# Autodesk Inventor assembly: Swingarm
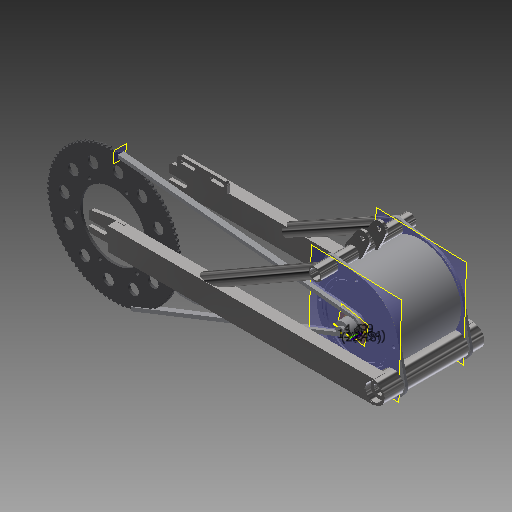
[picture p0: Inventor's stored thumbnail of the model, 512x512]
Saved by Autodesk Inventor 2019.3 (Build 233278000, 278)
## iProperties
Created: 2018-12-13
Part Number: Swingarm
Document SubType Name: Assembly
Designer: eroldan
Author: eroldan
## Documents named in this file (6)
- C:\Users\eroldan\Desktop\3dprojects\OpenEmoto\Swingarm3\Swingarm3.iam
- C:\Users\eroldan\Desktop\3dprojects\OpenEmoto\OtherParts\Denzel4500Motor.iam
- C:\Users\eroldan\Desktop\3dprojects\OpenEmoto\Swingarm3\Swingarm3.ipt
- C:\Users\eroldan\Desktop\3dprojects\OpenEmoto\OtherParts\Sprocket92T.ipt
- C:\Users\eroldan\Desktop\3dprojects\OpenEmoto\Swingarm3\BackMotorPlate.ipt
- C:\Users\eroldan\Desktop\3dprojects\OpenEmoto\Swingarm3\TestChain.ipt
## Components (6 placed, 5 different names)
1. Swingarm3:1 — Mate:2, Mate:3, Mate:4, Mate:5
2. Denzel4500Motor:1 [sub-assembly] — Mate:3, Flush:5, Flush:1, Flush:2, Flush:6, Mate:6
3. Sprocket92T:1 — Mate:2, Flush:5
4. BackMotorPlate:1 — Flush:1, Flush:2
5. TestChain:1 — Flush:6
6. BackMotorPlate:2 — Mate:4, Mate:5, Mate:6
## Relationships (9: Mate 5, Flush 4)
- Mate:2: Swingarm3:1 ↔ Sprocket92T:1
- Mate:3: Swingarm3:1 ↔ Denzel4500Motor:1
- Flush:5: Denzel4500Motor:1 ↔ Sprocket92T:1
- Flush:1: Denzel4500Motor:1 ↔ BackMotorPlate:1
- Flush:2: Denzel4500Motor:1 ↔ BackMotorPlate:1
- Flush:6: Denzel4500Motor:1 ↔ TestChain:1
- Mate:4: Swingarm3:1 ↔ BackMotorPlate:2
- Mate:5: Swingarm3:1 ↔ BackMotorPlate:2
- Mate:6: Denzel4500Motor:1 ↔ BackMotorPlate:2
